# Autodesk Inventor assembly: ArmsAssembly
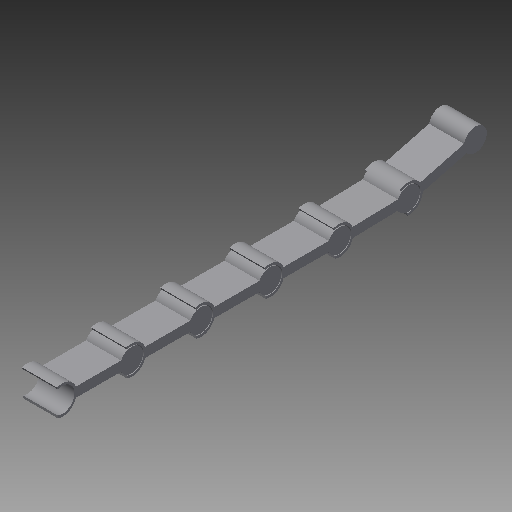
[picture p0: Inventor's stored thumbnail of the model, 512x512]
Saved by Autodesk Inventor 2018 (Build 220112000, 112)
## iProperties
Created: 2017-11-07
Part Number: ArmsAssembly
Document SubType Name: Assembly
Designer: kcmat
Author: kcmat
## Documents named in this file (2)
- C:\Users\reide\OneDrive\Documents\Inventor\TSA\2018\Animatronics\Tortoise\ArmsAssembly.iam
- C:\Users\reide\OneDrive\Documents\Inventor\TSA\2018\Animatronics\Tortoise\Legs\turtlearm.ipt
## Components (6 placed, 1 different names)
1. turtlearm:1 — Insert:1
2. turtlearm:2 — Insert:1, Insert:2
3. turtlearm:3 — Insert:2, Insert:3
4. turtlearm:4 — Insert:3, Insert:4
5. turtlearm:5 — Insert:4, Insert:5
6. turtlearm:6 — Insert:5
## Relationships (5: Insert 5)
- Insert:1: turtlearm:1 ↔ turtlearm:2
- Insert:2: turtlearm:2 ↔ turtlearm:3
- Insert:3: turtlearm:3 ↔ turtlearm:4
- Insert:4: turtlearm:4 ↔ turtlearm:5
- Insert:5: turtlearm:5 ↔ turtlearm:6
